# Autodesk Inventor assembly: parts_combined
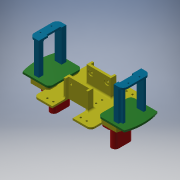
[picture p0: Inventor's stored thumbnail of the model, 180x180]
Saved by Autodesk Inventor 2016 (Build 200138000, 138)
## iProperties
Created: 2016-07-26
Part Number: parts_combined
Material: Générique
Document SubType Name: Assembly
Designer: tmonglon
Author: tmonglon
## Documents named in this file (5)
- D:\Inventor\Ahmet\ebug2014-chassis_2\pieces finies\parts_combined.iam
- D:\Inventor\Ahmet\ebug2014-chassis_2\pieces finies\yellow_part.ipt
- D:\Inventor\Ahmet\ebug2014-chassis_2\pieces finies\green_part.ipt
- D:\Inventor\Ahmet\ebug2014-chassis_2\pieces finies\Blue_part.ipt
- D:\Inventor\Ahmet\ebug2014-chassis_2\pieces finies\red_part.ipt
## Components (6 placed, 4 different names)
1. yellow_part:1 — Placage:1, Placage:2, Placage:3, Placage:4, Angle:1, Placage:5, Placage:6, Placage:7, Placage:8, Placage:9, Placage:10, Placage:13, Placage:14, Placage:15
2. green_part:1 — Placage:1, Placage:2, Placage:3, Placage:11
3. Blue_part:1 — Placage:4, Angle:1, Placage:5, Placage:6
4. red_part:1 — Placage:10, Placage:11, Placage:12
5. green_part:2 — Placage:7, Placage:8, Placage:9, Placage:12
6. Blue_part:2 — Placage:13, Placage:14, Placage:15
## Relationships (16: Mate 15, Angle 1)
- Placage:1 [Mate]: yellow_part:1 ↔ green_part:1
- Placage:2 [Mate]: yellow_part:1 ↔ green_part:1
- Placage:3 [Mate]: yellow_part:1 ↔ green_part:1
- Placage:4 [Mate]: yellow_part:1 ↔ Blue_part:1
- Angle:1 (0 deg): yellow_part:1 ↔ Blue_part:1
- Placage:5 [Mate]: yellow_part:1 ↔ Blue_part:1
- Placage:6 [Mate]: yellow_part:1 ↔ Blue_part:1
- Placage:7 [Mate]: yellow_part:1 ↔ green_part:2
- Placage:8 [Mate]: yellow_part:1 ↔ green_part:2
- Placage:9 [Mate]: yellow_part:1 ↔ green_part:2
- Placage:10 [Mate]: yellow_part:1 ↔ red_part:1
- Placage:11 [Mate]: green_part:1 ↔ red_part:1
- Placage:12 [Mate]: red_part:1 ↔ green_part:2
- Placage:13 [Mate]: yellow_part:1 ↔ Blue_part:2
- Placage:14 [Mate]: yellow_part:1 ↔ Blue_part:2
- Placage:15 [Mate]: yellow_part:1 ↔ Blue_part:2
